# Autodesk Inventor assembly: Pieza extra del mecanismo
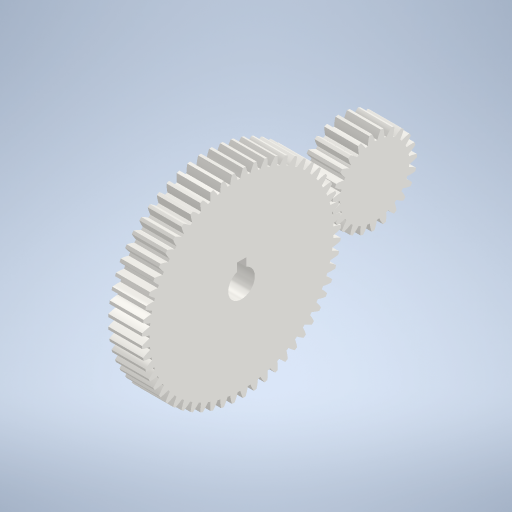
[picture p0: Inventor's stored thumbnail of the model, 512x512]
Saved by Autodesk Inventor 2024 (Build 280153000, 153)
## iProperties
Created: 2024-03-31
Part Number: Pieza extra del mecanismo
Document SubType Name: Assembly
Designer: darne
Author: darne
## Documents named in this file (6)
- C:\Users\darne\OneDrive\Escritorio\5to Semestre\Dinamica\Dinamica LAB\Pieza extra del mecanismo.iam
- C:\Users\darne\OneDrive\Escritorio\5to Semestre\Dinamica\Dinamica LAB\Mecanismo\CUÑA (1).ipt
- C:\Users\darne\OneDrive\Escritorio\5to Semestre\Dinamica\Dinamica LAB\Mecanismo\EJE_CUÑEROS.ipt
- C:\Users\darne\OneDrive\Escritorio\5to Semestre\Dinamica\Dinamica LAB\Mecanismo\ENGRANE.ipt
- C:\Users\darne\OneDrive\Escritorio\5to Semestre\Dinamica\Dinamica LAB\Mecanismo\POLEA.ipt
- C:\Users\darne\OneDrive\Escritorio\5to Semestre\Dinamica\Dinamica LAB\Mecanismo 1\Design Accelerator\Spur Gears1.iam
## Components (7 placed, 5 different names)
1. CUÑA (1):1 — Rigid:3, Mate:2, Planar:3
2. EJE_CUÑEROS:1 — Rigid:1, Flush:1, Rigid:2, Flush:2, Flush:3, Flush:4, Flush:5, Mate:1, Rigid:3, Mate:2, Planar:1, Rotational:1, Rotational:2, Rigid:4, Mate:3, Rotational:3, Rigid:5
3. ENGRANE:1 — Rigid:2, Flush:2, Flush:3, Flush:4, Flush:5, Mate:1, Flush:6, Mate:3, Rotational:3, Rigid:5
4. POLEA:1 — Rigid:1, Flush:1
5. CUÑA (1):2 — Planar:1
6. Spur Gears:1 [sub-assembly] — Rotational:1, Rotational:2, Rigid:4, Flush:6, Planar:2
7. CUÑA (1):3 — Planar:2, Planar:3
## Relationships (20: Flush 6, WeldJoint 5, Mate 3, PlanarJoint 3, RevoluteJoint 3)
- Rigid:1 [WeldJoint]: EJE_CUÑEROS:1 ↔ POLEA:1
- Flush:1: EJE_CUÑEROS:1 ↔ POLEA:1
- Rigid:2 [WeldJoint]: EJE_CUÑEROS:1 ↔ ENGRANE:1
- Flush:2 (0.127 mm): EJE_CUÑEROS:1 ↔ ENGRANE:1
- Flush:3 (-0.127 mm): EJE_CUÑEROS:1 ↔ ENGRANE:1
- Flush:4 (-25.4 mm): EJE_CUÑEROS:1 ↔ ENGRANE:1
- Flush:5 (25.4 mm): EJE_CUÑEROS:1 ↔ ENGRANE:1
- Mate:1 (0.127 mm): EJE_CUÑEROS:1 ↔ ENGRANE:1
- Rigid:3 [WeldJoint]: CUÑA (1):1 ↔ EJE_CUÑEROS:1
- Mate:2: CUÑA (1):1 ↔ EJE_CUÑEROS:1
- Planar:1: EJE_CUÑEROS:1 ↔ CUÑA (1):2
- Rotational:1 [RevoluteJoint]: EJE_CUÑEROS:1 ↔ Spur Gears:1
- Rotational:2 [RevoluteJoint]: EJE_CUÑEROS:1 ↔ Spur Gears:1
- Rigid:4 [WeldJoint]: EJE_CUÑEROS:1 ↔ Spur Gears:1
- Flush:6 (10 mm): ENGRANE:1 ↔ Spur Gears:1
- Mate:3 (10 mm): EJE_CUÑEROS:1 ↔ ENGRANE:1
- Rotational:3 [RevoluteJoint]: EJE_CUÑEROS:1 ↔ ENGRANE:1
- Rigid:5 [WeldJoint]: EJE_CUÑEROS:1 ↔ ENGRANE:1
- Planar:2: Spur Gears:1 ↔ CUÑA (1):3
- Planar:3: CUÑA (1):1 ↔ CUÑA (1):3
